# Autodesk Inventor assembly: Impulsor
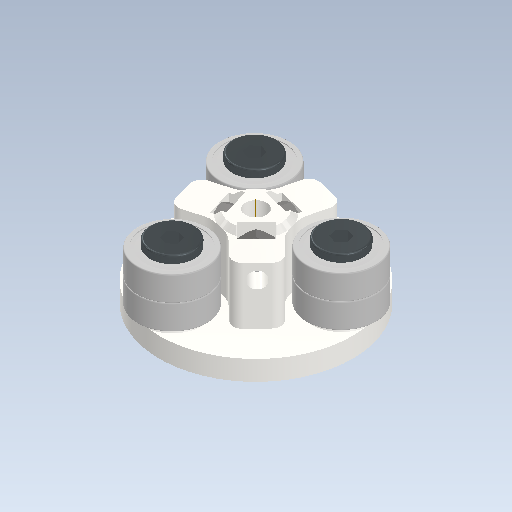
[picture p0: Inventor's stored thumbnail of the model, 512x512]
Saved by Autodesk Inventor 2020.2 (Build 242310000, 310)
## iProperties
Created: 2020-09-07
Part Number: Impulsor
Document SubType Name: Assembly
Designer: JK
Author: JK
## Documents named in this file (7)
- C:\Users\JK\Documents\Inventor\BioMixer\Sist dispensador de líquido viscoso\BombaPeristaltica\Impulsor.iam
- C:\Users\JK\Documents\Inventor\BioMixer\Sist dispensador de líquido viscoso\BombaPeristaltica\Impulsor.ipt
- C:\Users\JK\Documents\Inventor\BioMixer\Sist dispensador de líquido viscoso\BombaPeristaltica\TuercaM5BajoPerfil.ipt
- C:\Users\JK\Documents\Inventor\BioMixer\Sist dispensador de líquido viscoso\BombaPeristaltica\PrisioneroM3x6.ipt
- C:\Users\JK\Documents\Inventor\BioMixer\Sist dispensador de líquido viscoso\BombaPeristaltica\TuercaM3.ipt
- C:\Users\JK\Documents\Inventor\BioMixer\Sist dispensador de líquido viscoso\BombaPeristaltica\PernoM5x15Plano.ipt
- C:\Users\JK\Documents\Inventor\BioMixer\Sist dispensador de líquido viscoso\BombaPeristaltica\605ZZ\Rodamiento605ZZ.iam
## Components (19 placed, 6 different names)
1. Impulsor — Flush:5, Mate:22, Flush:6, Mate:37, Mate:40, Mate:42
2. Rodamiento605ZZ:1 [sub-assembly] — Mate:28, Mate:29, Mate:37
3. Rodamiento605ZZ:2 [sub-assembly] — Mate:28, Mate:29, Mate:40, Mate:41
4. PrisioneroM3x6:1 — Flush:6, Mate:43
5. TuercaM3:3 — Mate:22, Mate:42, Mate:43
6. TuercaM5BajoPerfil:1 — Mate:18, Flush:5
7. PernoM5x15Plano:3 — Mate:18, Mate:41
8. Rodamiento605ZZ:3 [sub-assembly]
9. Rodamiento605ZZ:4 [sub-assembly]
10. PrisioneroM3x6:2
11. TuercaM3:4
12. TuercaM5BajoPerfil:2
13. PernoM5x15Plano:4
14. Rodamiento605ZZ:5 [sub-assembly]
15. Rodamiento605ZZ:6 [sub-assembly]
16. PrisioneroM3x6:3
17. TuercaM3:5
18. TuercaM5BajoPerfil:3
19. PernoM5x15Plano:5
## Component patterns: (3 elements, first: Rodamiento605ZZ:1 + Rodamiento605ZZ:2 + PrisioneroM3x6:1 + TuercaM3:3 + TuercaM5BajoPerfil:1 + PernoM5x15Plano:3)
## Relationships (11: Mate 9, Flush 2)
- Mate:18: TuercaM5BajoPerfil:1 ↔ PernoM5x15Plano:3
- Flush:5: Impulsor ↔ TuercaM5BajoPerfil:1
- Mate:22: Impulsor ↔ TuercaM3:3
- Flush:6 (4 mm): Impulsor ↔ PrisioneroM3x6:1
- Mate:28: Rodamiento605ZZ:1 ↔ Rodamiento605ZZ:2
- Mate:29: Rodamiento605ZZ:1 ↔ Rodamiento605ZZ:2
- Mate:37: Impulsor ↔ Rodamiento605ZZ:1
- Mate:40: Impulsor ↔ Rodamiento605ZZ:2
- Mate:41: Rodamiento605ZZ:2 ↔ PernoM5x15Plano:3
- Mate:42: Impulsor ↔ TuercaM3:3
- Mate:43: PrisioneroM3x6:1 ↔ TuercaM3:3
